# Autodesk Inventor assembly: bb8 completo
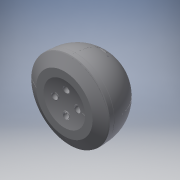
[picture p0: Inventor's stored thumbnail of the model, 180x180]
Saved by Autodesk Inventor 2016 (Build 200138000, 138)
## iProperties
Created: 2016-04-16
Part Number: bb8 completo
Material: Genérico
Document SubType Name: Assembly
Designer: Usuario1
Author: Usuario1
## Documents named in this file (5)
- C:\Users\Usuario1\Desktop\bb8 completo.iam
- C:\Users\Usuario1\Desktop\bb8_parte1.ipt
- C:\Users\Usuario1\Desktop\bb8_parte3.ipt
- C:\Users\Usuario1\Desktop\bb8_parte2.ipt
- C:\Users\Usuario1\Desktop\bb8_parte4.ipt
## Components (4 placed, 4 different names)
1. bb8_parte1:1 — Rígido:3, Rígido:5
2. bb8_parte2:1 — Rígido:3, Rígido:4
3. bb8_parte3:1 — Rígido:4
4. bb8_parte4:1 — Rígido:5
## Relationships (3: WeldJoint 3)
- Rígido:3 [WeldJoint]: bb8_parte1:1 ↔ bb8_parte2:1
- Rígido:4 [WeldJoint]: bb8_parte2:1 ↔ bb8_parte3:1
- Rígido:5 [WeldJoint]: bb8_parte1:1 ↔ bb8_parte4:1
